# Autodesk Inventor assembly: EL2-.100
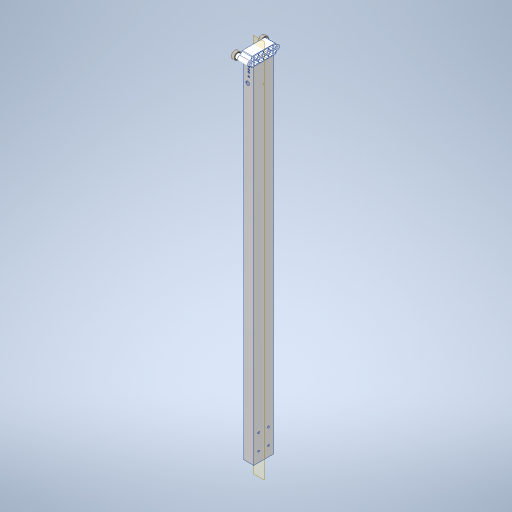
[picture p0: Inventor's stored thumbnail of the model, 512x512]
Saved by Autodesk Inventor 2023.4 (Build 274418000, 418)
## iProperties
Created: 2025-01-10
Part Number: EL2-.100
Document SubType Name: Assembly
Designer: mavericks
Author: mavericks
## Documents named in this file (4)
- C:\Users\mavericks\Desktop\2025-ReefScape---CAD\Elevator\EL2\EL2-.100.iam
- C:\Users\mavericks\Desktop\2025-ReefScape---CAD\Elevator\EL2\EL2-001.ipt
- C:\Users\mavericks\Desktop\2025-ReefScape---CAD\COMMON PARTS\WCP Elevator parts\WCP-0199\WCP-0199.iam
- C:\Users\mavericks\Desktop\2025-ReefScape---CAD\Elevator\EL2\EL2-400.iam
## Components (3 placed, 3 different names)
1. EL2-001:1 — Mate:1, Flush:1, Mate:2, Insert:1
2. WCP-0199:1 [sub-assembly] — Mate:1, Flush:1, Mate:2
3. EL2-400:1 [sub-assembly] — Insert:1
## Relationships (4: Mate 2, Flush 1, Insert 1)
- Mate:1: EL2-001:1 ↔ WCP-0199:1
- Flush:1: EL2-001:1 ↔ WCP-0199:1
- Mate:2: EL2-001:1 ↔ WCP-0199:1
- Insert:1: EL2-001:1 ↔ EL2-400:1
